# Autodesk Inventor assembly: High Strength Chain Generator
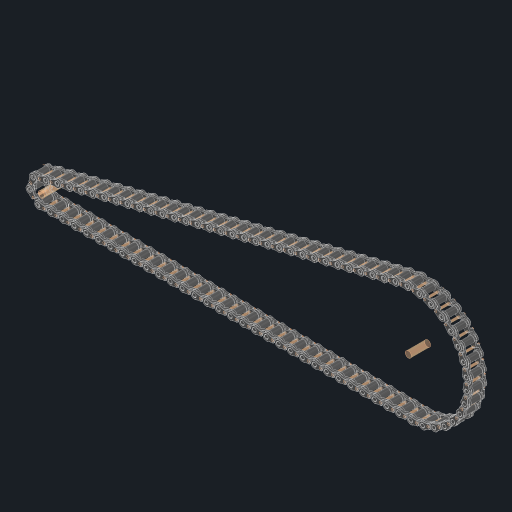
[picture p0: Inventor's stored thumbnail of the model, 512x512]
Saved by Autodesk Inventor 2023 (Build 270158000, 158)
## iProperties
RuleStatus: InUse
Created: 2020-07-07
Part Number: High Strength Chain Generator
Document SubType Name: Assembly
Designer: yuany
AfterDocOpen0: Open Form
Author: yuany
## Documents named in this file (3)
- C:\Users\ylu12\Documents\GitHub\VEX-CAD-Inventor\Motion\Chain Generator 9P\Chain Generator 9P.iam
- C:\Users\ylu12\Documents\GitHub\VEX-CAD-Inventor\Motion\Chain Generator 9P\Workpoint Pattern.ipt
- C:\Users\ylu12\Documents\GitHub\VEX-CAD-Inventor\Motion\Chain 9P\High Strength Chain Link.ipt
## Components (81 placed, 2 different names)
1. Workpoint Pattern:1 — Mate:1, Mate:2, Mate:3
2. High Strength Chain Link:1 — Mate:1, Mate:2, Mate:3
3. High Strength Chain Link:2
4. High Strength Chain Link:3
5. High Strength Chain Link:4
6. High Strength Chain Link:5
7. High Strength Chain Link:6
8. High Strength Chain Link:7
9. High Strength Chain Link:8
10. High Strength Chain Link:9
11. High Strength Chain Link:10
12. High Strength Chain Link:11
13. High Strength Chain Link:12
14. High Strength Chain Link:13
15. High Strength Chain Link:14
16. High Strength Chain Link:15
17. High Strength Chain Link:16
18. High Strength Chain Link:17
19. High Strength Chain Link:18
20. High Strength Chain Link:19
21. High Strength Chain Link:20
22. High Strength Chain Link:21
23. High Strength Chain Link:22
24. High Strength Chain Link:23
25. High Strength Chain Link:24
26. High Strength Chain Link:25
27. High Strength Chain Link:26
28. High Strength Chain Link:27
29. High Strength Chain Link:28
30. High Strength Chain Link:29
31. High Strength Chain Link:30
32. High Strength Chain Link:31
33. High Strength Chain Link:32
34. High Strength Chain Link:33
35. High Strength Chain Link:34
36. High Strength Chain Link:35
37. High Strength Chain Link:36
38. High Strength Chain Link:37
39. High Strength Chain Link:38
40. High Strength Chain Link:39
41. High Strength Chain Link:40
42. High Strength Chain Link:41
43. High Strength Chain Link:42
44. High Strength Chain Link:43
45. High Strength Chain Link:44
46. High Strength Chain Link:45
47. High Strength Chain Link:46
48. High Strength Chain Link:47
49. High Strength Chain Link:48
50. High Strength Chain Link:49
51. High Strength Chain Link:50
52. High Strength Chain Link:51
53. High Strength Chain Link:52
54. High Strength Chain Link:53
55. High Strength Chain Link:54
56. High Strength Chain Link:55
57. High Strength Chain Link:56
58. High Strength Chain Link:57
59. High Strength Chain Link:58
60. High Strength Chain Link:59
61. High Strength Chain Link:60
62. High Strength Chain Link:61
63. High Strength Chain Link:62
64. High Strength Chain Link:63
65. High Strength Chain Link:64
66. High Strength Chain Link:65
67. High Strength Chain Link:66
68. High Strength Chain Link:67
69. High Strength Chain Link:68
70. High Strength Chain Link:69
71. High Strength Chain Link:70
72. High Strength Chain Link:71
73. High Strength Chain Link:72
74. High Strength Chain Link:73
75. High Strength Chain Link:74
76. High Strength Chain Link:75
77. High Strength Chain Link:76
78. High Strength Chain Link:77
79. High Strength Chain Link:78
80. High Strength Chain Link:79
81. High Strength Chain Link:80
## Component patterns: (80 elements, first: High Strength Chain Link:1)
## Relationships (3: Mate 3)
- Mate:1: Workpoint Pattern:1 ↔ High Strength Chain Link:1
- Mate:2 (11.938 mm): Workpoint Pattern:1 ↔ High Strength Chain Link:1
- Mate:3: Workpoint Pattern:1 ↔ High Strength Chain Link:1
## Named parameters: Center_Distance = 304.8 mm, Sprocket1 = 19.558 mm, Sprocket2 = 93.726 mm, CenterDistance = 304.8 mm
